# Autodesk Inventor assembly: Leg_Loadpipe_Mount
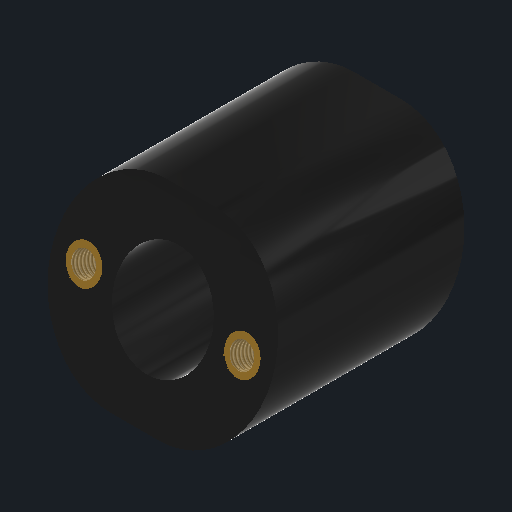
[picture p0: Inventor's stored thumbnail of the model, 512x512]
Saved by Autodesk Inventor 2024.1 (Build 281209000, 209)
## iProperties
Created: 2023-06-09
Part Number: Leg_Loadpipe_Mount
Document SubType Name: Assembly
Designer: dzw04
Author: dzw04
## Documents named in this file (4)
- C:\Users\dzw04\Saxion\Mechatronica Lectoraat LMECH LED - Database ARG\Component_Database\SARAX\01. CAD\01. 3D_Drawing\02. Sub_Assemblies\Landing_Gear\02. Sub_Assemblies\Leg_Loadpipe_Mount.iam
- C:\Users\dzw04\Saxion\Mechatronica Lectoraat LMECH LED - Database ARG\Component_Database\SARAX\01. CAD\01. 3D_Drawing\02. Sub_Assemblies\Landing_Gear\01. Parts\Leg_Loadpipe_Mount.ipt
- C:\Users\dzw04\Saxion\Mechatronica Lectoraat LMECH LED - Database ARG\Component_Database\SARAX\01. CAD\01. 3D_Drawing\01. Parts\Threaded_Insert_M3x4.ipt
- C:\Users\dzw04\OneDrive - Saxion\Documenten\Inventor\Content Center Files\R2024\en-US\DIN 913\DIN 913 - M4 x 4.ipt
## Components (7 placed, 3 different names)
1. Leg_Loadpipe_Mount:1 — Flush:1, Flush:2, Flush:3, Flush:4, Flush:5, Mate:1, Mate:2, Mate:3, Mate:4, Mate:5, Mate:6
2. Threaded_Insert_M3x4:1 — Flush:1, Mate:5
3. Threaded_Insert_M3x4:2 — Flush:2, Mate:4
4. Threaded_Insert_M3x4:3 — Flush:3, Mate:3
5. Threaded_Insert_M3x4:4 — Flush:5, Mate:1
6. Threaded_Insert_M3x4:5 — Flush:4, Mate:2
7. DIN 913 M4 x 4:1 — Mate:6
## Relationships (11: Mate 6, Flush 5)
- Flush:1: Leg_Loadpipe_Mount:1 ↔ Threaded_Insert_M3x4:1
- Flush:2: Leg_Loadpipe_Mount:1 ↔ Threaded_Insert_M3x4:2
- Flush:3: Leg_Loadpipe_Mount:1 ↔ Threaded_Insert_M3x4:3
- Flush:4: Leg_Loadpipe_Mount:1 ↔ Threaded_Insert_M3x4:5
- Flush:5: Leg_Loadpipe_Mount:1 ↔ Threaded_Insert_M3x4:4
- Mate:1: Leg_Loadpipe_Mount:1 ↔ Threaded_Insert_M3x4:4
- Mate:2: Leg_Loadpipe_Mount:1 ↔ Threaded_Insert_M3x4:5
- Mate:3: Leg_Loadpipe_Mount:1 ↔ Threaded_Insert_M3x4:3
- Mate:4: Leg_Loadpipe_Mount:1 ↔ Threaded_Insert_M3x4:2
- Mate:5: Leg_Loadpipe_Mount:1 ↔ Threaded_Insert_M3x4:1
- Mate:6: Leg_Loadpipe_Mount:1 ↔ DIN 913 M4 x 4:1
